# Autodesk Inventor assembly: CuboidSecurityBoxCovered
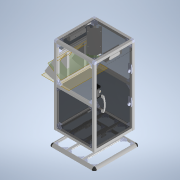
[picture p0: Inventor's stored thumbnail of the model, 180x180]
Saved by Autodesk Inventor 2021.3 (Build 253353000, 353)
## iProperties
Created: 2020-11-09
Part Number: CuboidSecurityBoxCovered
Document SubType Name: Assembly
Designer: gisen
Author: gisen
## Documents named in this file (13)
- C:\Users\gisen\GitProjects\CAD-Data\CuboidAccessories\SecurityBox\CuboidSecurityBoxCoveredTypeB.iam
- C:\Users\gisen\GitProjects\CAD-Data\CuboidAccessories\SecurityBox\Assemblies\CuboidSecurityBoxBasisTypeB.iam
- C:\Users\gisen\GitProjects\CAD-Data\GeneralComponentsTemplate\Fittings\BasicFrameBracket.ipt
- C:\Users\gisen\GitProjects\CAD-Data\CuboidAccessories\SecurityBox\Frames\BasicFrameCornerSide290.ipt
- C:\Users\gisen\GitProjects\CAD-Data\CuboidAccessories\SecurityBox\Plates\OutsideTopPlate.ipt
- C:\Users\gisen\GitProjects\CAD-Data\CuboidAccessories\CuboidTopFrame\CuboidTopFrame.iam
- C:\Users\gisen\GitProjects\CAD-Data\Devices\SolenoidLatch\SolenoidLatchAssembly.iam
- C:\Users\gisen\GitProjects\CAD-Data\GeneralComponentsTemplate\Hinges\Hinge-DHS-3239.iam
- C:\Users\gisen\GitProjects\CAD-Data\CuboidAccessories\SecurityBox\Assemblies\DoorAssembly.iam
- C:\Users\gisen\GitProjects\CAD-Data\Devices\RealSenseD435\RealSenseD543Assembly.iam
- C:\Users\gisen\GitProjects\CAD-Data\CuboidAccessories\SecurityBox\Plates\DoorPlateUpper.ipt
- C:\Users\gisen\GitProjects\CAD-Data\CuboidAccessories\SecurityBox\3DPrintedParts\CableCover.ipt
- C:\Users\gisen\GitProjects\CAD-Data\CuboidAccessories\SecurityBox\3DPrintedParts\CableCoverForFrame.ipt
## Components (20 placed, 12 different names)
1. CuboidSecurityBoxBasisTypeB:1 [sub-assembly] — フラッシュ:1, フラッシュ:2, メイト:1, メイト:2, メイト:3, メイト:4, メイト:5, メイト:6, メイト:7, メイト:9, メイト:12, メイト:13, フラッシュ:3, メイト:14, フラッシュ:4, フラッシュ:5, フラッシュ:6, メイト:18, メイト:19, メイト:20, メイト:22, メイト:23, フラッシュ:7, フラッシュ:8, メイト:31, メイト:36, メイト:37, メイト:39, メイト:42, フラッシュ:9, メイト:43, メイト:44, メイト:45, メイト:48, メイト:49, メイト:50, メイト:51, メイト:52, メイト:53
2. BasicFrameBracket:1 — メイト:11, メイト:12, メイト:13
3. BasicFrameCornerSide290:1 — フラッシュ:1, フラッシュ:2, メイト:1, メイト:8, メイト:10, メイト:11, メイト:15, メイト:21, メイト:25, メイト:29, メイト:30, メイト:35, メイト:38, メイト:40, メイト:41
4. BasicFrameBracket:2 — メイト:8, メイト:9, メイト:10
5. BasicFrameBracket:3 — メイト:5, メイト:6, メイト:7
6. BasicFrameBracket:4 — メイト:2, メイト:3, メイト:4
7. OutsideTopPlate:1 — フラッシュ:3, メイト:14, メイト:15, メイト:46, メイト:47, フラッシュ:10
8. CuboidTopFrame:1 [sub-assembly] — メイト:16, メイト:17
9. SolenoidLatchAssembly:1 [sub-assembly] — メイト:18, メイト:19, メイト:25
10. Hinge-DHS-3239:1 [sub-assembly] — メイト:20, メイト:21, フラッシュ:8, メイト:32, メイト:34
11. Hinge-DHS-3239:2 [sub-assembly] — メイト:22, メイト:23, フラッシュ:7, メイト:33
12. DoorAssembly:1 [sub-assembly] — メイト:32, メイト:33, メイト:34
13. RealSenseD543Assembly:1 [sub-assembly] — メイト:29, メイト:30, メイト:31
14. DoorPlateUpper:1 — メイト:41, メイト:42, フラッシュ:9
15. BasicFrameBracket:5 — メイト:35, メイト:36, メイト:37
16. BasicFrameBracket:6 — メイト:38, メイト:39, メイト:40
17. RealSenseD543Assembly:2 [sub-assembly] — メイト:43, メイト:44, メイト:45
18. CableCover:1 — メイト:46, メイト:47, フラッシュ:10
19. CableCoverForFrame:1 — メイト:48, メイト:49, メイト:53
20. CableCoverForFrame:2 — メイト:50, メイト:51, メイト:52
## Relationships (59: Mate 49, Flush 10)
- フラッシュ:1 [Flush]: CuboidSecurityBoxBasisTypeB:1 ↔ BasicFrameCornerSide290:1
- フラッシュ:2 [Flush]: CuboidSecurityBoxBasisTypeB:1 ↔ BasicFrameCornerSide290:1
- メイト:1 [Mate]: CuboidSecurityBoxBasisTypeB:1 ↔ BasicFrameCornerSide290:1
- メイト:2 [Mate]: CuboidSecurityBoxBasisTypeB:1 ↔ BasicFrameBracket:4
- メイト:3 [Mate] (-10 mm): CuboidSecurityBoxBasisTypeB:1 ↔ BasicFrameBracket:4
- メイト:4 [Mate]: CuboidSecurityBoxBasisTypeB:1 ↔ BasicFrameBracket:4
- メイト:5 [Mate]: CuboidSecurityBoxBasisTypeB:1 ↔ BasicFrameBracket:3
- メイト:6 [Mate] (-10 mm): CuboidSecurityBoxBasisTypeB:1 ↔ BasicFrameBracket:3
- メイト:7 [Mate]: CuboidSecurityBoxBasisTypeB:1 ↔ BasicFrameBracket:3
- メイト:8 [Mate]: BasicFrameCornerSide290:1 ↔ BasicFrameBracket:2
- メイト:9 [Mate]: CuboidSecurityBoxBasisTypeB:1 ↔ BasicFrameBracket:2
- メイト:10 [Mate] (-10 mm): BasicFrameCornerSide290:1 ↔ BasicFrameBracket:2
- メイト:11 [Mate]: BasicFrameBracket:1 ↔ BasicFrameCornerSide290:1
- メイト:12 [Mate]: CuboidSecurityBoxBasisTypeB:1 ↔ BasicFrameBracket:1
- メイト:13 [Mate] (-10 mm): CuboidSecurityBoxBasisTypeB:1 ↔ BasicFrameBracket:1
- フラッシュ:3 [Flush]: CuboidSecurityBoxBasisTypeB:1 ↔ OutsideTopPlate:1
- メイト:14 [Mate]: CuboidSecurityBoxBasisTypeB:1 ↔ OutsideTopPlate:1
- メイト:15 [Mate]: BasicFrameCornerSide290:1 ↔ OutsideTopPlate:1
- フラッシュ:4 [Flush]: CuboidSecurityBoxBasisTypeB:1
- フラッシュ:5 [Flush]: CuboidSecurityBoxBasisTypeB:1
- フラッシュ:6 [Flush]: CuboidSecurityBoxBasisTypeB:1
- メイト:16 [Mate]: CuboidTopFrame:1
- メイト:17 [Mate]: CuboidTopFrame:1
- メイト:18 [Mate]: CuboidSecurityBoxBasisTypeB:1 ↔ SolenoidLatchAssembly:1
- メイト:19 [Mate]: CuboidSecurityBoxBasisTypeB:1 ↔ SolenoidLatchAssembly:1
- メイト:20 [Mate]: CuboidSecurityBoxBasisTypeB:1 ↔ Hinge-DHS-3239:1
- メイト:21 [Mate] (150 mm): BasicFrameCornerSide290:1 ↔ Hinge-DHS-3239:1
- メイト:22 [Mate]: CuboidSecurityBoxBasisTypeB:1 ↔ Hinge-DHS-3239:2
- メイト:23 [Mate] (150 mm): CuboidSecurityBoxBasisTypeB:1 ↔ Hinge-DHS-3239:2
- メイト:25 [Mate] (210 mm): BasicFrameCornerSide290:1 ↔ SolenoidLatchAssembly:1
- フラッシュ:7 [Flush]: CuboidSecurityBoxBasisTypeB:1 ↔ Hinge-DHS-3239:2
- フラッシュ:8 [Flush]: CuboidSecurityBoxBasisTypeB:1 ↔ Hinge-DHS-3239:1
- メイト:29 [Mate]: BasicFrameCornerSide290:1 ↔ RealSenseD543Assembly:1
- メイト:30 [Mate]: BasicFrameCornerSide290:1 ↔ RealSenseD543Assembly:1
- メイト:31 [Mate] (80 mm): CuboidSecurityBoxBasisTypeB:1 ↔ RealSenseD543Assembly:1
- メイト:32 [Mate]: Hinge-DHS-3239:1 ↔ DoorAssembly:1
- メイト:33 [Mate]: Hinge-DHS-3239:2 ↔ DoorAssembly:1
- メイト:34 [Mate]: Hinge-DHS-3239:1 ↔ DoorAssembly:1
- メイト:35 [Mate]: BasicFrameCornerSide290:1 ↔ BasicFrameBracket:5
- メイト:36 [Mate]: CuboidSecurityBoxBasisTypeB:1 ↔ BasicFrameBracket:5
- メイト:37 [Mate] (-10 mm): CuboidSecurityBoxBasisTypeB:1 ↔ BasicFrameBracket:5
- メイト:38 [Mate]: BasicFrameCornerSide290:1 ↔ BasicFrameBracket:6
- メイト:39 [Mate]: CuboidSecurityBoxBasisTypeB:1 ↔ BasicFrameBracket:6
- メイト:40 [Mate] (-10 mm): BasicFrameCornerSide290:1 ↔ BasicFrameBracket:6
- メイト:41 [Mate]: BasicFrameCornerSide290:1 ↔ DoorPlateUpper:1
- メイト:42 [Mate]: CuboidSecurityBoxBasisTypeB:1 ↔ DoorPlateUpper:1
- フラッシュ:9 [Flush]: CuboidSecurityBoxBasisTypeB:1 ↔ DoorPlateUpper:1
- メイト:43 [Mate]: CuboidSecurityBoxBasisTypeB:1 ↔ RealSenseD543Assembly:2
- メイト:44 [Mate]: CuboidSecurityBoxBasisTypeB:1 ↔ RealSenseD543Assembly:2
- メイト:45 [Mate] (80 mm): CuboidSecurityBoxBasisTypeB:1 ↔ RealSenseD543Assembly:2
- メイト:46 [Mate]: OutsideTopPlate:1 ↔ CableCover:1
- メイト:47 [Mate]: OutsideTopPlate:1 ↔ CableCover:1
- フラッシュ:10 [Flush]: OutsideTopPlate:1 ↔ CableCover:1
- メイト:48 [Mate]: CuboidSecurityBoxBasisTypeB:1 ↔ CableCoverForFrame:1
- メイト:49 [Mate]: CuboidSecurityBoxBasisTypeB:1 ↔ CableCoverForFrame:1
- メイト:50 [Mate]: CuboidSecurityBoxBasisTypeB:1 ↔ CableCoverForFrame:2
- メイト:51 [Mate]: CuboidSecurityBoxBasisTypeB:1 ↔ CableCoverForFrame:2
- メイト:52 [Mate] (50 mm): CuboidSecurityBoxBasisTypeB:1 ↔ CableCoverForFrame:2
- メイト:53 [Mate] (50 mm): CuboidSecurityBoxBasisTypeB:1 ↔ CableCoverForFrame:1
